# Autodesk Inventor assembly: Ensamblaje1-Polea
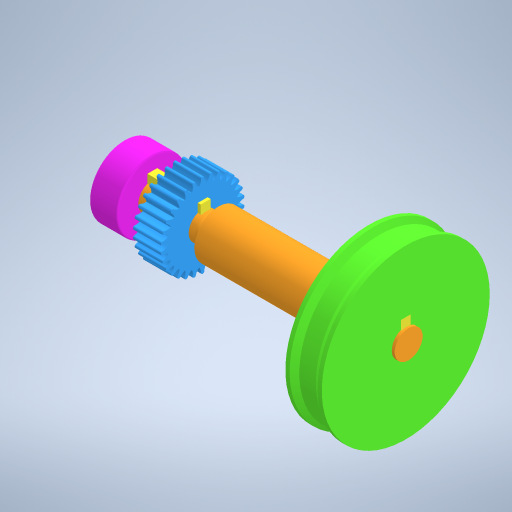
[picture p0: Inventor's stored thumbnail of the model, 512x512]
Saved by Autodesk Inventor 2024 (Build 280153000, 153)
## iProperties
Created: 2024-03-28
Part Number: Ensamblaje1-Polea
Document SubType Name: Assembly
Designer: kelly
Author: kelly
## Documents named in this file (6)
- C:\Users\kelly\OneDrive\Documentos\2024\Dinámica - Lab\Ensamblaje1-Polea.iam
- C:\Users\kelly\Downloads\EJE_CUÑEROS.ipt
- C:\Users\kelly\Downloads\PIEZA PARA GIRAR.ipt
- C:\Users\kelly\Downloads\POLEA.ipt
- C:\Users\kelly\Downloads\ENGRANE.ipt
- C:\Users\kelly\Downloads\CUÑA.ipt
## Components (7 placed, 5 different names)
1. EJE_CUÑEROS:1 — Rígido:1, Rígido:2, Rígido:3, Rígido:5, Rígido:6, Rígido:7
2. PIEZA PARA GIRAR:1 — Rígido:6
3. POLEA:1 — Rígido:7
4. ENGRANE:1 — Rígido:5
5. CUÑA:1 — Rígido:3
6. CUÑA:2 — Rígido:2
7. CUÑA:3 — Rígido:1
## Relationships (6: WeldJoint 6)
- Rígido:1 [WeldJoint]: EJE_CUÑEROS:1 ↔ CUÑA:3
- Rígido:2 [WeldJoint]: EJE_CUÑEROS:1 ↔ CUÑA:2
- Rígido:3 [WeldJoint]: EJE_CUÑEROS:1 ↔ CUÑA:1
- Rígido:5 [WeldJoint] (-56 mm): EJE_CUÑEROS:1 ↔ ENGRANE:1
- Rígido:6 [WeldJoint]: EJE_CUÑEROS:1 ↔ PIEZA PARA GIRAR:1
- Rígido:7 [WeldJoint] (-2.08 mm): EJE_CUÑEROS:1 ↔ POLEA:1
